# Autodesk Inventor assembly: 夹体
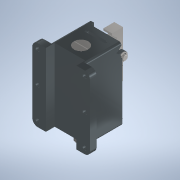
[picture p0: Inventor's stored thumbnail of the model, 180x180]
Saved by Autodesk Inventor 2022 (Build 260153000, 153)
## iProperties
Created: 2023-01-14
Part Number: 夹体
Document SubType Name: Assembly
Designer: Lzy18
Author: Lzy18
## Documents named in this file (10)
- C:\Users\Lzy18\Desktop\夹体\夹体.iam
- C:\Users\Lzy18\Desktop\夹体\1-夹具体.ipt
- C:\Users\Lzy18\Desktop\夹体\部件1.iam
- C:\Users\Lzy18\Desktop\夹体\4-上盖.ipt
- C:\Users\Lzy18\Desktop\夹体\部件2.iam
- C:\Users\Lzy18\Desktop\夹体\5-压铁.ipt
- C:\Users\Lzy18\Desktop\夹体\6-鞘轴.ipt
- C:\Users\Lzy18\Desktop\夹体\11-垫圈.ipt
- C:\Users\Lzy18\Desktop\夹体\13-螺钉.ipt
- C:\Users\Lzy18\Documents\Inventor\Content Center Files\R2022\zh-CN\ASME B27.8M(2)\ASME B27.8M - 3EM1-11.ipt
## Components (13 placed, 9 different names)
1. 1-夹具体:1 — 插入:1, 配合:1, 配合:2, 配合:3, 配合:11
2. 部件1:1 [sub-assembly] — 插入:1, 角度:2
3. 4-上盖:1 — 配合:1, 配合:2, 配合:3, 配合:4, 配合:5, 配合:6, 插入:2, 插入:3, 插入:4, 插入:5, 插入:6, 角度:1, 角度:2, 配合:12
4. 部件2:1 [sub-assembly] — 配合:4, 配合:11
5. 5-压铁:1 — 配合:5, 配合:6, 配合:7, 配合:8, 配合:9, 配合:10, 角度:1
6. 6-鞘轴:1 — 插入:2, 配合:13
7. 11-垫圈:1 — 配合:7, 配合:8
8. 11-垫圈:2 — 配合:9, 配合:10
9. 13-螺钉:1 — 插入:4
10. 13-螺钉:2 — 插入:3
11. 13-螺钉:3 — 插入:6
12. 13-螺钉:4 — 插入:5
13. ASME B27.8M 3EM1-11:1 — 配合:12, 配合:13
## Relationships (21: Mate 13, Insert 6, Angle 2)
- 插入:1 [Insert]: 1-夹具体:1 ↔ 部件1:1
- 配合:1 [Mate]: 1-夹具体:1 ↔ 4-上盖:1
- 配合:2 [Mate]: 1-夹具体:1 ↔ 4-上盖:1
- 配合:3 [Mate]: 1-夹具体:1 ↔ 4-上盖:1
- 配合:4 [Mate]: 4-上盖:1 ↔ 部件2:1
- 配合:5 [Mate] (2 mm): 4-上盖:1 ↔ 5-压铁:1
- 配合:6 [Mate] (2 mm): 4-上盖:1 ↔ 5-压铁:1
- 插入:2 [Insert]: 4-上盖:1 ↔ 6-鞘轴:1
- 配合:7 [Mate]: 5-压铁:1 ↔ 11-垫圈:1
- 配合:8 [Mate]: 5-压铁:1 ↔ 11-垫圈:1
- 配合:9 [Mate]: 5-压铁:1 ↔ 11-垫圈:2
- 配合:10 [Mate]: 5-压铁:1 ↔ 11-垫圈:2
- 插入:3 [Insert]: 4-上盖:1 ↔ 13-螺钉:2
- 插入:4 [Insert]: 4-上盖:1 ↔ 13-螺钉:1
- 插入:5 [Insert]: 4-上盖:1 ↔ 13-螺钉:4
- 插入:6 [Insert]: 4-上盖:1 ↔ 13-螺钉:3
- 角度:1 [Angle] (0 deg): 4-上盖:1 ↔ 5-压铁:1
- 配合:11 [Mate]: 1-夹具体:1 ↔ 部件2:1
- 角度:2 [Angle] (0 deg): 部件1:1 ↔ 4-上盖:1
- 配合:12 [Mate]: 4-上盖:1 ↔ ASME B27.8M 3EM1-11:1
- 配合:13 [Mate]: 6-鞘轴:1 ↔ ASME B27.8M 3EM1-11:1
